# Autodesk Inventor assembly: antana
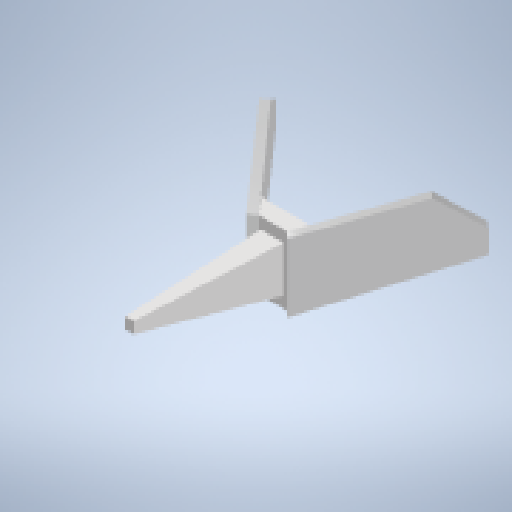
[picture p0: Inventor's stored thumbnail of the model, 512x512]
Saved by Autodesk Inventor 2024.1 (Build 281209000, 209)
## iProperties
Created: 2024-02-25
Part Number: antana
Document SubType Name: Assembly
Designer: hibik
Author: hibik
## Documents named in this file (4)
- C:\Users\hibik\Desktop\ロボメカ\HR\2024.02.11 Rl\02.11 ProtType\head\antana.iam
- C:\Users\hibik\Desktop\ロボメカ\HR\2024.02.11 Rl\02.11 ProtType\head\antana_middle.ipt
- C:\Users\hibik\Desktop\ロボメカ\HR\2024.02.11 Rl\02.11 ProtType\head\antana_side.ipt
- C:\Users\hibik\Desktop\ロボメカ\HR\2024.02.11 Rl\02.11 ProtType\head\amtana.ipt
## Components (4 placed, 3 different names)
1. antana_middle:1 — メイト:1, メイト:2, メイト:3, メイト:4, メイト:5, メイト:6, メイト:7, フラッシュ:1
2. antana_side:1 — メイト:1, メイト:3, メイト:5
3. antana_side:2 — メイト:2, メイト:4, メイト:6
4. amtana:1 — メイト:7, フラッシュ:1
## Relationships (8: Mate 7, Flush 1)
- メイト:1 [Mate]: antana_middle:1 ↔ antana_side:1
- メイト:2 [Mate]: antana_middle:1 ↔ antana_side:2
- メイト:3 [Mate]: antana_middle:1 ↔ antana_side:1
- メイト:4 [Mate]: antana_middle:1 ↔ antana_side:2
- メイト:5 [Mate]: antana_middle:1 ↔ antana_side:1
- メイト:6 [Mate]: antana_middle:1 ↔ antana_side:2
- メイト:7 [Mate]: antana_middle:1 ↔ amtana:1
- フラッシュ:1 [Flush] (2 mm): antana_middle:1 ↔ amtana:1
